# Autodesk Inventor assembly: 全体アセンブリ
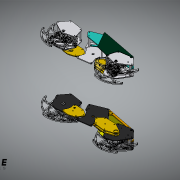
[picture p0: Inventor's stored thumbnail of the model, 180x180]
Saved by Autodesk Inventor 2019 (Build 230136000, 136)
## iProperties
Created: 2019-09-17
Part Number: 全体アセンブリ
Material: 一般
Document SubType Name: Assembly
Designer: tanjihayato
Author: tanjihayato
## Documents named in this file (41)
- \\Mac\Home\Documents\Inventor\2019お遊び機体\全体アセンブリ.iam
- \\Mac\Home\Documents\Inventor\2019お遊び機体\前足内フレーム.ipt
- \\Mac\Home\Documents\Inventor\2019お遊び機体\新型３クランクアセンブリ.iam
- \\Mac\Home\Documents\Inventor\2019お遊び機体\新型３脚最終段カム.ipt
- \\Mac\Home\Documents\Inventor\2019お遊び機体\スペーサ　m3-l35.ipt
- \\Mac\Home\Documents\Inventor\2019お遊び機体\新型３ヘッケン.ipt
- \\Mac\Home\Documents\Inventor\2019お遊び機体\新型３揺動節.ipt
- \\Mac\Home\Documents\Inventor\2019お遊び機体\線図.ipt
- \\Mac\Home\Documents\Inventor\2019お遊び機体\中間内フレーム.ipt
- \\Mac\Home\Documents\Inventor\2019お遊び機体\台形サスバー.ipt
- \\Mac\Home\Documents\Inventor\2019お遊び機体\ギアトレイン.ipt
- \\Mac\Home\Documents\Inventor\2019お遊び機体\スペーサ　m3-l5.ipt
- \\Mac\Home\Documents\Inventor\2019お遊び機体\中間外フレーム.ipt
- \\Mac\Home\Documents\Inventor\2019お遊び機体\前足外フレーム.ipt
- \\Mac\Home\Documents\Inventor\2019お遊び機体\前足カバー.ipt
- \\Mac\Home\Documents\Inventor\2019お遊び機体\後ろ脚内フレーム.ipt
- \\Mac\Home\Documents\Inventor\2019お遊び機体\後ろ脚内フレーム２.ipt
- \\Mac\Home\Documents\Inventor\2019お遊び機体\新型３クランクアセンブリ_MIR.iam
- \\Mac\Home\Documents\Inventor\2019お遊び機体\新型３ヘッケン_MIR.ipt
- \\Mac\Home\Documents\Inventor\2019お遊び機体\新型３揺動節_MIR.ipt
- \\Mac\Home\Documents\Inventor\2019お遊び機体\後ろ脚外フレーム.ipt
- \\Mac\Home\Documents\Inventor\2019お遊び機体\前足内フレーム_MIR.ipt
- \\Mac\Home\Documents\Inventor\2019お遊び機体\新型３クランクアセンブリ_MIR1.iam
- \\Mac\Home\Documents\Inventor\2019お遊び機体\新型３脚最終段カム_MIR.ipt
- \\Mac\Home\Documents\Inventor\2019お遊び機体\スペーサ　m3-l35_MIR.ipt
- \\Mac\Home\Documents\Inventor\2019お遊び機体\新型３ヘッケン_MIR1.ipt
- \\Mac\Home\Documents\Inventor\2019お遊び機体\新型３揺動節_MIR1.ipt
- \\Mac\Home\Documents\Inventor\2019お遊び機体\中間内フレーム_MIR.ipt
- \\Mac\Home\Documents\Inventor\2019お遊び機体\台形サスバー_MIR.ipt
- \\Mac\Home\Documents\Inventor\2019お遊び機体\ギアトレイン_MIR.ipt
- \\Mac\Home\Documents\Inventor\2019お遊び機体\スペーサ　m3-l5_MIR.ipt
- \\Mac\Home\Documents\Inventor\2019お遊び機体\中間外フレーム_MIR.ipt
- \\Mac\Home\Documents\Inventor\2019お遊び機体\前足外フレーム_MIR.ipt
- \\Mac\Home\Documents\Inventor\2019お遊び機体\前足カバー_MIR.ipt
- \\Mac\Home\Documents\Inventor\2019お遊び機体\後ろ脚内フレーム_MIR.ipt
- \\Mac\Home\Documents\Inventor\2019お遊び機体\後ろ脚内フレーム２_MIR.ipt
- \\Mac\Home\Documents\Inventor\2019お遊び機体\新型３クランクアセンブリ_MIR_MIR.iam
- \\Mac\Home\Documents\Inventor\2019お遊び機体\新型３ヘッケン_MIR_MIR.ipt
- \\Mac\Home\Documents\Inventor\2019お遊び機体\新型３揺動節_MIR_MIR.ipt
- \\Mac\Home\Documents\Inventor\2019お遊び機体\後ろ脚外フレーム_MIR.ipt
- \\Mac\Home\Documents\Inventor\2019お遊び機体\台形サスバー板.ipt
## Components (103 placed, 40 different names)
1. 前足内フレーム:1 — 挿入:29, 挿入:31, 挿入:32, 挿入:33, 挿入:37, 挿入:38
2. 新型３クランクアセンブリ:1 [sub-assembly] — 挿入:1, メイト:1, 挿入:8, 挿入:9, 挿入:10, 挿入:11
3. 新型３脚最終段カム:1 — 挿入:1, メイト:1, 挿入:38
4. スペーサ　m3-l35:1 — 挿入:31, 挿入:34, 挿入:35
5. スペーサ　m3-l35:2 — 挿入:29
6. スペーサ　m3-l35:3 — 挿入:33, 挿入:39
7. スペーサ　m3-l35:4 — メイト:2, メイト:3, メイト:4, メイト:5, 挿入:32, メイト:15
8. 新型３ヘッケン:1 — 挿入:11, 挿入:14
9. 新型３ヘッケン:2 — 挿入:10, 挿入:13
10. 新型３ヘッケン:3 — 挿入:9, 挿入:12
11. 新型３ヘッケン:4 — 挿入:7, 挿入:8
12. 新型３揺動節:1 — メイト:2, 挿入:7
13. 新型３揺動節:2 — メイト:3, 挿入:13
14. 新型３揺動節:3 — メイト:4, 挿入:12
15. 新型３揺動節:4 — メイト:5, 挿入:14
16. 線図:1 — メイト:11, メイト:12, メイト:13
17. 中間内フレーム:1 — メイト:11, メイト:12, メイト:13, 挿入:22, 挿入:23, 挿入:24, 挿入:25, 挿入:36, 挿入:42
18. 台形サスバー:1 — 挿入:27, 挿入:34, メイト:41
19. 台形サスバー:2 — 挿入:28, 挿入:35, メイト:42, フラッシュ:1
20. ギアトレイン:1 — 挿入:15, 挿入:16, 挿入:17, 挿入:18, 挿入:19, 挿入:20
21. ギアトレイン:2 — 挿入:21, メイト:10, 挿入:36, 挿入:37
22. スペーサ　m3-l5:1 — 挿入:17
23. スペーサ　m3-l5:2 — 挿入:20, メイト:10
24. スペーサ　m3-l5:3 — 挿入:19
25. スペーサ　m3-l5:4 — 挿入:16
26. スペーサ　m3-l5:5 — 挿入:15, 挿入:21
27. スペーサ　m3-l5:6 — 挿入:18
28. スペーサ　m3-l35:5 — 挿入:22, 挿入:26, 挿入:27, 挿入:28, メイト:40
29. スペーサ　m3-l35:6 — 挿入:23, メイト:14
30. スペーサ　m3-l35:7 — 挿入:25
31. スペーサ　m3-l35:8 — 挿入:24
32. 中間外フレーム:1 — 挿入:26, メイト:14, 挿入:109
33. 前足外フレーム:1 — 挿入:39, メイト:15, 挿入:40, メイト:16
34. 前足カバー:1 — 挿入:40, メイト:16
35. 後ろ脚内フレーム:1 — 挿入:41, メイト:17, 挿入:42
36. 後ろ脚内フレーム２:1 — 挿入:41, メイト:17, 挿入:51, 挿入:52, 挿入:53, 挿入:54, 挿入:56
37. 新型３クランクアセンブリ_MIR:1 [sub-assembly] — 挿入:43, 挿入:44, 挿入:45, 挿入:46, 挿入:55, メイト:18
38. 新型３ヘッケン_MIR:1 — 挿入:43, 挿入:50
39. 新型３ヘッケン_MIR:2 — 挿入:44, 挿入:48
40. 新型３ヘッケン_MIR:3 — 挿入:45, 挿入:49
41. 新型３ヘッケン_MIR:4 — 挿入:46, 挿入:47
42. 新型３揺動節_MIR:1 — 挿入:47, メイト:20
43. 新型３揺動節_MIR:2 — 挿入:48, メイト:22
44. 新型３揺動節_MIR:3 — 挿入:49, メイト:21
45. 新型３揺動節_MIR:4 — 挿入:50, メイト:19
46. スペーサ　m3-l35:9 — 挿入:52, メイト:23
47. スペーサ　m3-l35:10 — 挿入:51
48. スペーサ　m3-l35:11 — 挿入:54, メイト:19, メイト:20, メイト:21, メイト:22, 挿入:57
49. スペーサ　m3-l35:12 — 挿入:53
50. 新型３脚最終段カム:2 — 挿入:55, メイト:18, 挿入:56
51. 後ろ脚外フレーム:1 — 挿入:57, メイト:23
52. 前足内フレーム_MIR:1 — 挿入:58, 挿入:60, 挿入:61, 挿入:62, 挿入:63, 挿入:74
53. 新型３クランクアセンブリ_MIR1:1 [sub-assembly] — メイト:24, 挿入:59, 挿入:64, 挿入:65, 挿入:66, 挿入:67
54. 新型３脚最終段カム_MIR:1 — 挿入:58, メイト:24, 挿入:59
55. スペーサ　m3-l35_MIR:1 — 挿入:60, 挿入:72, 挿入:73
56. スペーサ　m3-l35_MIR:2 — 挿入:61
57. スペーサ　m3-l35_MIR:3 — 挿入:62, 挿入:90
58. スペーサ　m3-l35_MIR:4 — 挿入:63, メイト:25, メイト:26, メイト:27, メイト:28, メイト:31
59. 新型３ヘッケン_MIR1:1 — 挿入:64, 挿入:71
60. 新型３ヘッケン_MIR1:2 — 挿入:65, 挿入:69
61. 新型３ヘッケン_MIR1:3 — 挿入:66, 挿入:70
62. 新型３ヘッケン_MIR1:4 — 挿入:67, 挿入:68
63. 新型３揺動節_MIR1:1 — 挿入:68, メイト:25
64. 新型３揺動節_MIR1:2 — 挿入:69, メイト:26
65. 新型３揺動節_MIR1:3 — 挿入:70, メイト:27
66. 新型３揺動節_MIR1:4 — 挿入:71, メイト:28
67. 中間内フレーム_MIR:1 — 挿入:75, 挿入:85, 挿入:86, 挿入:87, 挿入:88, 挿入:92
68. 台形サスバー_MIR:1 — 挿入:72, 挿入:84, メイト:44, フラッシュ:2
69. 台形サスバー_MIR:2 — 挿入:73, 挿入:83, メイト:43
70. ギアトレイン_MIR:1 — 挿入:76, 挿入:77, 挿入:78, 挿入:79, 挿入:81, 挿入:82
71. ギアトレイン_MIR:2 — 挿入:74, 挿入:75, メイト:29, 挿入:80
72. スペーサ　m3-l5_MIR:1 — 挿入:76
73. スペーサ　m3-l5_MIR:2 — メイト:29, 挿入:77
74. スペーサ　m3-l5_MIR:3 — 挿入:78
75. スペーサ　m3-l5_MIR:4 — 挿入:79
76. スペーサ　m3-l5_MIR:5 — 挿入:80, 挿入:81
77. スペーサ　m3-l5_MIR:6 — 挿入:82
78. スペーサ　m3-l35_MIR:5 — 挿入:83, 挿入:84, 挿入:85, 挿入:89
79. スペーサ　m3-l35_MIR:6 — 挿入:86, メイト:30
80. スペーサ　m3-l35_MIR:7 — 挿入:87
81. スペーサ　m3-l35_MIR:8 — 挿入:88
82. 中間外フレーム_MIR:1 — メイト:30, 挿入:89, 挿入:109, メイト:40
83. 前足外フレーム_MIR:1 — メイト:31, 挿入:90, メイト:32, 挿入:91
84. 前足カバー_MIR:1 — メイト:32, 挿入:91
85. 後ろ脚内フレーム_MIR:1 — 挿入:92, メイト:33, 挿入:93
86. 後ろ脚内フレーム２_MIR:1 — メイト:33, 挿入:93, 挿入:102, 挿入:103, 挿入:104, 挿入:105, 挿入:106
87. 新型３クランクアセンブリ_MIR_MIR:1 [sub-assembly] — 挿入:94, 挿入:95, 挿入:96, 挿入:97, メイト:38, 挿入:107
88. 新型３ヘッケン_MIR_MIR:1 — 挿入:94, 挿入:101
89. 新型３ヘッケン_MIR_MIR:2 — 挿入:95, 挿入:99
90. 新型３ヘッケン_MIR_MIR:3 — 挿入:96, 挿入:100
91. 新型３ヘッケン_MIR_MIR:4 — 挿入:97, 挿入:98
92. 新型３揺動節_MIR_MIR:1 — 挿入:98, メイト:36
93. 新型３揺動節_MIR_MIR:2 — 挿入:99, メイト:34
94. 新型３揺動節_MIR_MIR:3 — 挿入:100, メイト:35
95. 新型３揺動節_MIR_MIR:4 — 挿入:101, メイト:37
96. スペーサ　m3-l35_MIR:9 — 挿入:102, メイト:39
97. スペーサ　m3-l35_MIR:10 — 挿入:103
98. スペーサ　m3-l35_MIR:11 — メイト:34, メイト:35, メイト:36, メイト:37, 挿入:104, 挿入:108
99. スペーサ　m3-l35_MIR:12 — 挿入:105
100. 新型３脚最終段カム_MIR:2 — 挿入:106, メイト:38, 挿入:107
101. 後ろ脚外フレーム_MIR:1 — メイト:39, 挿入:108
102. 台形サスバー板:1 — メイト:41, メイト:42, フラッシュ:1
103. 台形サスバー板:2 — メイト:43, メイト:44, フラッシュ:2
## Relationships (145: Insert 103, Mate 40, Flush 2)
- 挿入:1 [Insert]: 新型３クランクアセンブリ:1 ↔ 新型３脚最終段カム:1
- メイト:1 [Mate]: 新型３クランクアセンブリ:1 ↔ 新型３脚最終段カム:1
- メイト:2 [Mate]: スペーサ　m3-l35:4 ↔ 新型３揺動節:1
- メイト:3 [Mate]: スペーサ　m3-l35:4 ↔ 新型３揺動節:2
- メイト:4 [Mate]: スペーサ　m3-l35:4 ↔ 新型３揺動節:3
- メイト:5 [Mate]: スペーサ　m3-l35:4 ↔ 新型３揺動節:4
- 挿入:7 [Insert]: 新型３ヘッケン:4 ↔ 新型３揺動節:1
- 挿入:8 [Insert] (0.25 mm): 新型３クランクアセンブリ:1 ↔ 新型３ヘッケン:4
- 挿入:9 [Insert] (0.25 mm): 新型３クランクアセンブリ:1 ↔ 新型３ヘッケン:3
- 挿入:10 [Insert] (0.25 mm): 新型３クランクアセンブリ:1 ↔ 新型３ヘッケン:2
- 挿入:11 [Insert] (0.25 mm): 新型３クランクアセンブリ:1 ↔ 新型３ヘッケン:1
- 挿入:12 [Insert]: 新型３ヘッケン:3 ↔ 新型３揺動節:3
- 挿入:13 [Insert]: 新型３ヘッケン:2 ↔ 新型３揺動節:2
- 挿入:14 [Insert]: 新型３ヘッケン:1 ↔ 新型３揺動節:4
- 挿入:15 [Insert]: ギアトレイン:1 ↔ スペーサ　m3-l5:5
- 挿入:16 [Insert]: ギアトレイン:1 ↔ スペーサ　m3-l5:4
- 挿入:17 [Insert]: ギアトレイン:1 ↔ スペーサ　m3-l5:1
- 挿入:18 [Insert]: ギアトレイン:1 ↔ スペーサ　m3-l5:6
- 挿入:19 [Insert]: ギアトレイン:1 ↔ スペーサ　m3-l5:3
- 挿入:20 [Insert]: ギアトレイン:1 ↔ スペーサ　m3-l5:2
- 挿入:21 [Insert]: ギアトレイン:2 ↔ スペーサ　m3-l5:5
- メイト:10 [Mate]: ギアトレイン:2 ↔ スペーサ　m3-l5:2
- メイト:11 [Mate]: 線図:1 ↔ 中間内フレーム:1
- メイト:12 [Mate]: 線図:1 ↔ 中間内フレーム:1
- メイト:13 [Mate]: 線図:1 ↔ 中間内フレーム:1
- 挿入:22 [Insert]: 中間内フレーム:1 ↔ スペーサ　m3-l35:5
- 挿入:23 [Insert]: 中間内フレーム:1 ↔ スペーサ　m3-l35:6
- 挿入:24 [Insert]: 中間内フレーム:1 ↔ スペーサ　m3-l35:8
- 挿入:25 [Insert]: 中間内フレーム:1 ↔ スペーサ　m3-l35:7
- 挿入:26 [Insert]: スペーサ　m3-l35:5 ↔ 中間外フレーム:1
- メイト:14 [Mate]: スペーサ　m3-l35:6 ↔ 中間外フレーム:1
- 挿入:27 [Insert]: 台形サスバー:1 ↔ スペーサ　m3-l35:5
- 挿入:28 [Insert]: 台形サスバー:2 ↔ スペーサ　m3-l35:5
- 挿入:29 [Insert]: 前足内フレーム:1 ↔ スペーサ　m3-l35:2
- 挿入:31 [Insert]: 前足内フレーム:1 ↔ スペーサ　m3-l35:1
- 挿入:32 [Insert]: 前足内フレーム:1 ↔ スペーサ　m3-l35:4
- 挿入:33 [Insert]: 前足内フレーム:1 ↔ スペーサ　m3-l35:3
- 挿入:34 [Insert]: スペーサ　m3-l35:1 ↔ 台形サスバー:1
- 挿入:35 [Insert]: スペーサ　m3-l35:1 ↔ 台形サスバー:2
- 挿入:36 [Insert]: 中間内フレーム:1 ↔ ギアトレイン:2
- 挿入:37 [Insert]: 前足内フレーム:1 ↔ ギアトレイン:2
- 挿入:38 [Insert] (-0.5 mm): 前足内フレーム:1 ↔ 新型３脚最終段カム:1
- 挿入:39 [Insert]: スペーサ　m3-l35:3 ↔ 前足外フレーム:1
- メイト:15 [Mate]: スペーサ　m3-l35:4 ↔ 前足外フレーム:1
- 挿入:40 [Insert]: 前足外フレーム:1 ↔ 前足カバー:1
- メイト:16 [Mate]: 前足外フレーム:1 ↔ 前足カバー:1
- 挿入:41 [Insert]: 後ろ脚内フレーム:1 ↔ 後ろ脚内フレーム２:1
- メイト:17 [Mate]: 後ろ脚内フレーム:1 ↔ 後ろ脚内フレーム２:1
- 挿入:42 [Insert]: 中間内フレーム:1 ↔ 後ろ脚内フレーム:1
- 挿入:43 [Insert] (0.25 mm): 新型３クランクアセンブリ_MIR:1 ↔ 新型３ヘッケン_MIR:1
- 挿入:44 [Insert] (0.25 mm): 新型３クランクアセンブリ_MIR:1 ↔ 新型３ヘッケン_MIR:2
- 挿入:45 [Insert] (0.25 mm): 新型３クランクアセンブリ_MIR:1 ↔ 新型３ヘッケン_MIR:3
- 挿入:46 [Insert] (0.25 mm): 新型３クランクアセンブリ_MIR:1 ↔ 新型３ヘッケン_MIR:4
- 挿入:47 [Insert]: 新型３ヘッケン_MIR:4 ↔ 新型３揺動節_MIR:1
- 挿入:48 [Insert]: 新型３ヘッケン_MIR:2 ↔ 新型３揺動節_MIR:2
- 挿入:49 [Insert]: 新型３ヘッケン_MIR:3 ↔ 新型３揺動節_MIR:3
- 挿入:50 [Insert]: 新型３ヘッケン_MIR:1 ↔ 新型３揺動節_MIR:4
- 挿入:51 [Insert]: 後ろ脚内フレーム２:1 ↔ スペーサ　m3-l35:10
- 挿入:52 [Insert]: 後ろ脚内フレーム２:1 ↔ スペーサ　m3-l35:9
- 挿入:53 [Insert]: 後ろ脚内フレーム２:1 ↔ スペーサ　m3-l35:12
- 挿入:54 [Insert]: 後ろ脚内フレーム２:1 ↔ スペーサ　m3-l35:11
- 挿入:55 [Insert]: 新型３クランクアセンブリ_MIR:1 ↔ 新型３脚最終段カム:2
- メイト:18 [Mate]: 新型３クランクアセンブリ_MIR:1 ↔ 新型３脚最終段カム:2
- 挿入:56 [Insert]: 後ろ脚内フレーム２:1 ↔ 新型３脚最終段カム:2
- メイト:19 [Mate]: 新型３揺動節_MIR:4 ↔ スペーサ　m3-l35:11
- メイト:20 [Mate]: 新型３揺動節_MIR:1 ↔ スペーサ　m3-l35:11
- メイト:21 [Mate]: 新型３揺動節_MIR:3 ↔ スペーサ　m3-l35:11
- メイト:22 [Mate]: 新型３揺動節_MIR:2 ↔ スペーサ　m3-l35:11
- 挿入:57 [Insert]: スペーサ　m3-l35:11 ↔ 後ろ脚外フレーム:1
- メイト:23 [Mate]: スペーサ　m3-l35:9 ↔ 後ろ脚外フレーム:1
- 挿入:58 [Insert] (-0.5 mm): 前足内フレーム_MIR:1 ↔ 新型３脚最終段カム_MIR:1
- メイト:24 [Mate]: 新型３クランクアセンブリ_MIR1:1 ↔ 新型３脚最終段カム_MIR:1
- 挿入:59 [Insert]: 新型３クランクアセンブリ_MIR1:1 ↔ 新型３脚最終段カム_MIR:1
- 挿入:60 [Insert]: 前足内フレーム_MIR:1 ↔ スペーサ　m3-l35_MIR:1
- 挿入:61 [Insert]: 前足内フレーム_MIR:1 ↔ スペーサ　m3-l35_MIR:2
- 挿入:62 [Insert]: 前足内フレーム_MIR:1 ↔ スペーサ　m3-l35_MIR:3
- 挿入:63 [Insert]: 前足内フレーム_MIR:1 ↔ スペーサ　m3-l35_MIR:4
- 挿入:64 [Insert] (0.25 mm): 新型３クランクアセンブリ_MIR1:1 ↔ 新型３ヘッケン_MIR1:1
- 挿入:65 [Insert] (0.25 mm): 新型３クランクアセンブリ_MIR1:1 ↔ 新型３ヘッケン_MIR1:2
- 挿入:66 [Insert] (0.25 mm): 新型３クランクアセンブリ_MIR1:1 ↔ 新型３ヘッケン_MIR1:3
- 挿入:67 [Insert] (0.25 mm): 新型３クランクアセンブリ_MIR1:1 ↔ 新型３ヘッケン_MIR1:4
- 挿入:68 [Insert]: 新型３ヘッケン_MIR1:4 ↔ 新型３揺動節_MIR1:1
- メイト:25 [Mate]: スペーサ　m3-l35_MIR:4 ↔ 新型３揺動節_MIR1:1
- 挿入:69 [Insert]: 新型３ヘッケン_MIR1:2 ↔ 新型３揺動節_MIR1:2
- メイト:26 [Mate]: スペーサ　m3-l35_MIR:4 ↔ 新型３揺動節_MIR1:2
- 挿入:70 [Insert]: 新型３ヘッケン_MIR1:3 ↔ 新型３揺動節_MIR1:3
- メイト:27 [Mate]: スペーサ　m3-l35_MIR:4 ↔ 新型３揺動節_MIR1:3
- 挿入:71 [Insert]: 新型３ヘッケン_MIR1:1 ↔ 新型３揺動節_MIR1:4
- メイト:28 [Mate]: スペーサ　m3-l35_MIR:4 ↔ 新型３揺動節_MIR1:4
- 挿入:72 [Insert]: スペーサ　m3-l35_MIR:1 ↔ 台形サスバー_MIR:1
- 挿入:73 [Insert]: スペーサ　m3-l35_MIR:1 ↔ 台形サスバー_MIR:2
- 挿入:74 [Insert]: 前足内フレーム_MIR:1 ↔ ギアトレイン_MIR:2
- 挿入:75 [Insert]: 中間内フレーム_MIR:1 ↔ ギアトレイン_MIR:2
- 挿入:76 [Insert]: ギアトレイン_MIR:1 ↔ スペーサ　m3-l5_MIR:1
- メイト:29 [Mate]: ギアトレイン_MIR:2 ↔ スペーサ　m3-l5_MIR:2
- 挿入:77 [Insert]: ギアトレイン_MIR:1 ↔ スペーサ　m3-l5_MIR:2
- 挿入:78 [Insert]: ギアトレイン_MIR:1 ↔ スペーサ　m3-l5_MIR:3
- 挿入:79 [Insert]: ギアトレイン_MIR:1 ↔ スペーサ　m3-l5_MIR:4
- 挿入:80 [Insert]: ギアトレイン_MIR:2 ↔ スペーサ　m3-l5_MIR:5
- 挿入:81 [Insert]: ギアトレイン_MIR:1 ↔ スペーサ　m3-l5_MIR:5
- 挿入:82 [Insert]: ギアトレイン_MIR:1 ↔ スペーサ　m3-l5_MIR:6
- 挿入:83 [Insert]: 台形サスバー_MIR:2 ↔ スペーサ　m3-l35_MIR:5
- 挿入:84 [Insert]: 台形サスバー_MIR:1 ↔ スペーサ　m3-l35_MIR:5
- 挿入:85 [Insert]: 中間内フレーム_MIR:1 ↔ スペーサ　m3-l35_MIR:5
- 挿入:86 [Insert]: 中間内フレーム_MIR:1 ↔ スペーサ　m3-l35_MIR:6
- 挿入:87 [Insert]: 中間内フレーム_MIR:1 ↔ スペーサ　m3-l35_MIR:7
- 挿入:88 [Insert]: 中間内フレーム_MIR:1 ↔ スペーサ　m3-l35_MIR:8
- メイト:30 [Mate]: スペーサ　m3-l35_MIR:6 ↔ 中間外フレーム_MIR:1
- 挿入:89 [Insert]: スペーサ　m3-l35_MIR:5 ↔ 中間外フレーム_MIR:1
- メイト:31 [Mate]: スペーサ　m3-l35_MIR:4 ↔ 前足外フレーム_MIR:1
- 挿入:90 [Insert]: スペーサ　m3-l35_MIR:3 ↔ 前足外フレーム_MIR:1
- メイト:32 [Mate]: 前足外フレーム_MIR:1 ↔ 前足カバー_MIR:1
- 挿入:91 [Insert]: 前足外フレーム_MIR:1 ↔ 前足カバー_MIR:1
- 挿入:92 [Insert]: 中間内フレーム_MIR:1 ↔ 後ろ脚内フレーム_MIR:1
- メイト:33 [Mate]: 後ろ脚内フレーム_MIR:1 ↔ 後ろ脚内フレーム２_MIR:1
- 挿入:93 [Insert]: 後ろ脚内フレーム_MIR:1 ↔ 後ろ脚内フレーム２_MIR:1
- 挿入:94 [Insert] (0.25 mm): 新型３クランクアセンブリ_MIR_MIR:1 ↔ 新型３ヘッケン_MIR_MIR:1
- 挿入:95 [Insert] (0.25 mm): 新型３クランクアセンブリ_MIR_MIR:1 ↔ 新型３ヘッケン_MIR_MIR:2
- 挿入:96 [Insert] (0.25 mm): 新型３クランクアセンブリ_MIR_MIR:1 ↔ 新型３ヘッケン_MIR_MIR:3
- 挿入:97 [Insert] (0.25 mm): 新型３クランクアセンブリ_MIR_MIR:1 ↔ 新型３ヘッケン_MIR_MIR:4
- 挿入:98 [Insert]: 新型３ヘッケン_MIR_MIR:4 ↔ 新型３揺動節_MIR_MIR:1
- 挿入:99 [Insert]: 新型３ヘッケン_MIR_MIR:2 ↔ 新型３揺動節_MIR_MIR:2
- 挿入:100 [Insert]: 新型３ヘッケン_MIR_MIR:3 ↔ 新型３揺動節_MIR_MIR:3
- 挿入:101 [Insert]: 新型３ヘッケン_MIR_MIR:1 ↔ 新型３揺動節_MIR_MIR:4
- 挿入:102 [Insert]: 後ろ脚内フレーム２_MIR:1 ↔ スペーサ　m3-l35_MIR:9
- 挿入:103 [Insert]: 後ろ脚内フレーム２_MIR:1 ↔ スペーサ　m3-l35_MIR:10
- メイト:34 [Mate]: 新型３揺動節_MIR_MIR:2 ↔ スペーサ　m3-l35_MIR:11
- メイト:35 [Mate]: 新型３揺動節_MIR_MIR:3 ↔ スペーサ　m3-l35_MIR:11
- メイト:36 [Mate]: 新型３揺動節_MIR_MIR:1 ↔ スペーサ　m3-l35_MIR:11
- メイト:37 [Mate]: 新型３揺動節_MIR_MIR:4 ↔ スペーサ　m3-l35_MIR:11
- 挿入:104 [Insert]: 後ろ脚内フレーム２_MIR:1 ↔ スペーサ　m3-l35_MIR:11
- 挿入:105 [Insert]: 後ろ脚内フレーム２_MIR:1 ↔ スペーサ　m3-l35_MIR:12
- 挿入:106 [Insert]: 後ろ脚内フレーム２_MIR:1 ↔ 新型３脚最終段カム_MIR:2
- メイト:38 [Mate]: 新型３クランクアセンブリ_MIR_MIR:1 ↔ 新型３脚最終段カム_MIR:2
- 挿入:107 [Insert]: 新型３クランクアセンブリ_MIR_MIR:1 ↔ 新型３脚最終段カム_MIR:2
- メイト:39 [Mate]: スペーサ　m3-l35_MIR:9 ↔ 後ろ脚外フレーム_MIR:1
- 挿入:108 [Insert]: スペーサ　m3-l35_MIR:11 ↔ 後ろ脚外フレーム_MIR:1
- 挿入:109 [Insert] (-300 mm): 中間外フレーム:1 ↔ 中間外フレーム_MIR:1
- メイト:40 [Mate]: スペーサ　m3-l35:5 ↔ 中間外フレーム_MIR:1
- メイト:41 [Mate]: 台形サスバー:1 ↔ 台形サスバー板:1
- メイト:42 [Mate]: 台形サスバー:2 ↔ 台形サスバー板:1
- フラッシュ:1 [Flush]: 台形サスバー:2 ↔ 台形サスバー板:1
- メイト:43 [Mate]: 台形サスバー_MIR:2 ↔ 台形サスバー板:2
- メイト:44 [Mate]: 台形サスバー_MIR:1 ↔ 台形サスバー板:2
- フラッシュ:2 [Flush]: 台形サスバー_MIR:1 ↔ 台形サスバー板:2
